# Autodesk Inventor assembly: totmannschalter
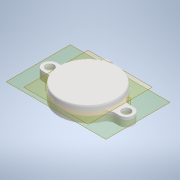
[picture p0: Inventor's stored thumbnail of the model, 180x180]
Saved by Autodesk Inventor 2021.3 (Build 253353010, 353A)
## iProperties
Created: 2021-08-03
Part Number: totmannschalter
Document SubType Name: Assembly
Designer: Markus
Author: Markus
## Documents named in this file (3)
- C:\Users\Markus\Documents\Inventor\MotorController\totmannschalter.iam
- C:\Users\Markus\Documents\Inventor\MotorController\totmannschalter_grundplatte.ipt
- C:\Users\Markus\Documents\Inventor\MotorController\totmannschalter_deckel.ipt
## Components (2 placed, 2 different names)
1. totmannschalter_grundplatte:1 — Fluchtend:1, Fluchtend:2
2. totmannschalter_deckel:1 — Fluchtend:1, Fluchtend:2
## Relationships (2: Flush 2)
- Fluchtend:1 [Flush]: totmannschalter_grundplatte:1 ↔ totmannschalter_deckel:1
- Fluchtend:2 [Flush]: totmannschalter_grundplatte:1 ↔ totmannschalter_deckel:1
